# Autodesk Inventor assembly: EnsamblajeMoto
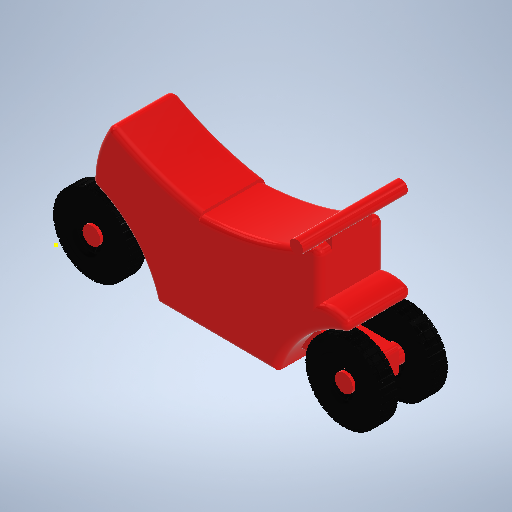
[picture p0: Inventor's stored thumbnail of the model, 512x512]
Saved by Autodesk Inventor 2025.2 (Build 292293000, 293)
## iProperties
Created: 2025-01-19
Part Number: EnsamblajeMoto
Document SubType Name: Assembly
Designer: usuario
Author: usuario
## Documents named in this file (4)
- C:\Users\usuario\Desktop\ModeladosAPM\MOTO\EnsamblajeMoto.iam
- C:\Users\usuario\Desktop\ModeladosAPM\MOTO\PiezaParteAtrasMoto.ipt
- C:\Users\usuario\Desktop\ModeladosAPM\MOTO\Llanta.ipt
- C:\Users\usuario\Desktop\ModeladosAPM\MOTO\PiezaParteDelanteraMoto.ipt
## Components (6 placed, 3 different names)
1. PiezaParteAtrasMoto:1 — Coincidencia:1, Nivelación:1, Nivelación:2, Coincidencia:2, Nivelación:3, Coincidencia:4, Nivelación:5
2. Llanta:1 — Coincidencia:2, Nivelación:3
3. Llanta:2 — Coincidencia:3, Nivelación:4
4. Llanta:3 — Coincidencia:5, Nivelación:6
5. Llanta:4 — Coincidencia:4, Nivelación:5
6. PiezaParteDelanteraMoto:1 — Coincidencia:1, Nivelación:1, Nivelación:2, Coincidencia:3, Nivelación:4, Coincidencia:5, Nivelación:6
## Relationships (11: Flush 6, Mate 5)
- Coincidencia:1 [Mate]: PiezaParteAtrasMoto:1 ↔ PiezaParteDelanteraMoto:1
- Nivelación:1 [Flush]: PiezaParteAtrasMoto:1 ↔ PiezaParteDelanteraMoto:1
- Nivelación:2 [Flush]: PiezaParteAtrasMoto:1 ↔ PiezaParteDelanteraMoto:1
- Coincidencia:2 [Mate]: PiezaParteAtrasMoto:1 ↔ Llanta:1
- Nivelación:3 [Flush]: PiezaParteAtrasMoto:1 ↔ Llanta:1
- Coincidencia:3 [Mate]: Llanta:2 ↔ PiezaParteDelanteraMoto:1
- Nivelación:4 [Flush]: Llanta:2 ↔ PiezaParteDelanteraMoto:1
- Coincidencia:4 [Mate]: PiezaParteAtrasMoto:1 ↔ Llanta:4
- Nivelación:5 [Flush]: PiezaParteAtrasMoto:1 ↔ Llanta:4
- Coincidencia:5 [Mate]: Llanta:3 ↔ PiezaParteDelanteraMoto:1
- Nivelación:6 [Flush]: Llanta:3 ↔ PiezaParteDelanteraMoto:1
